# Autodesk Inventor assembly: MOR-20C-6-10
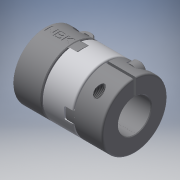
[picture p0: Inventor's stored thumbnail of the model, 180x180]
Saved by Autodesk Inventor 2019 (Build 230136000, 136)
## iProperties
Category: PARTsolutions
Company: NBK
Created: 2024-03-13
Part Number: MOR-20C-6-10
Catalog Web Link: www.cadenas.de
Description: MOR-C-
Vendor: NBK
Document SubType Name: Assembly
Designer: psAdmin
Manufacturer: NBK
Mass: 6.20778 g
Surface Area: 44.699 cm^2
Volume: 6.20778 cm^3
Density: 1 g/cm^3
Title: MOR-20C-6-10
Author: Cadenas PARTsolutions
PSOL_IDENT_0: {$CADENAS_DATA/23d-libs/nbk/motion_control_parts/couplicon_mini/oldham_type/mor/mor_c_asmtab.prj},18
PSOL_IDENT_1: 2 {VTYP=3D},{STYP=ASSTAB},{NB=MOR-20C-6-10},{LINA=MOR-20C-6-10},{NN=MOR-C},{DATE=12.03.2024 08:53:07
PSOL_IDENT_2: },{GEOMDATE=13.12.2021 11:44:02},{VERSION=},{LINEID=240},{WBVAR=D1D2},{WBNUMERIC=}  {NB=MOR-20C-6-10
PSOL_IDENT_3: },{LINA=MOR-20C-6-10},{KT=DUMMY},{CN=MOR-20C},{D1D2=6-10},{A=20},{L=8.8},{W=27.6},{E=12.2},{F=4.4},{
PSOL_IDENT_4: G=7.5},{M=M3},{WT=1.5},{D1D2X1='5-5','5-6','5-6.35','5-8','5-9.525','5-10','6-6','6-6.35','6-8','6-9
PSOL_IDENT_5: .525','6-10','6.35-6.35','6.35-8','6.35-9.525','6.35-10','8-8','8-9.525','8-10','9.525-9.525','9.525
PSOL_IDENT_6: -10','10-10','1/4-1/4','1/4-5/16','1/4-3/8','5/16-5/16','5/16-3/8','3/8-3/8','5-1/4','5-5/16','5-3/8'
PSOL_IDENT_7: ,'6-1/4','6-5/16','6-3/8','6.35-1/4','6.35-5/16','6.35-3/8','8-3/8','9.525-3/8','1/4-8','1/4-9.525','
PSOL_IDENT_8: 1/4-10','5/16-8','5/16-9.525','5/16-10','3/8-10'},{D1=6},{D2=10},{PPATH=mor_c_asmtpl.prj},{CNSORDERN
PSOL_IDENT_9: O=MOR-20C-6-10}
NB: MOR-20C-6-10
NN: MOR-C
NBSYN: $CN.-$D1D2.
LINA: MOR-20C-6-10
CATALOG: NBK (Nabeya Bi-tech Kaisha
CN: MOR-20C
D1D2: 6-10
A: 20
L: 8.8
W: 27.6
E: 12.2
F: 4.4
G: 7.5
M: M3
WT: 1.5
SUPPLIER: NBK
ARTICLENO: MOR-20C-6-10
BOMINFO: MOR-20C-6-10
CREATOR: CADENAS GmbH
## Documents named in this file (4)
- e:\temp\worker_COMMON_2\temp\tmp_7396_62_syEQ4\format_0\MOR-20C-6-10.iam
- e:\temp\worker_COMMON_2\temp\tmp_7396_62_syEQ4\format_0\MOR-20C - 6-10 Hub 1.ipt
- e:\temp\worker_COMMON_2\temp\tmp_7396_62_syEQ4\format_0\MOR-20C  Sleeve.ipt
- e:\temp\worker_COMMON_2\temp\tmp_7396_62_syEQ4\format_0\MOR-20C - 6-10 Hub 2.ipt
## Components (3 placed, 3 different names)
1. MOR-20C - 6-10 Hub 1:1 — p1_p2_XY@1 <-> p2_p1_XY@2, p1_p2_Z@1 <-> p2_p1_Z@2, p1_p2_YZ@1 <-> p2_p1_YZ@2
2. MOR-20C  Sleeve:1 — p1_p2_XY@1 <-> p2_p1_XY@2, p1_p2_Z@1 <-> p2_p1_Z@2, p1_p2_YZ@1 <-> p2_p1_YZ@2, p2_p3_XY@2 <-> p3_p2_XY@3, p2_p3_Z@2 <-> p3_p2_Z@3, p2_p3_YZ@2 <-> p3_p2_YZ@3
3. MOR-20C - 6-10 Hub 2:1 — p2_p3_XY@2 <-> p3_p2_XY@3, p2_p3_Z@2 <-> p3_p2_Z@3, p2_p3_YZ@2 <-> p3_p2_YZ@3
## Relationships (6: Mate 4, Angle 2)
- p1_p2_XY@1 <-> p2_p1_XY@2 [Mate]: MOR-20C - 6-10 Hub 1:1 ↔ MOR-20C  Sleeve:1
- p1_p2_Z@1 <-> p2_p1_Z@2 [Mate]: MOR-20C - 6-10 Hub 1:1 ↔ MOR-20C  Sleeve:1
- p1_p2_YZ@1 <-> p2_p1_YZ@2 [Angle] (0 deg): MOR-20C - 6-10 Hub 1:1 ↔ MOR-20C  Sleeve:1
- p2_p3_XY@2 <-> p3_p2_XY@3 [Mate]: MOR-20C  Sleeve:1 ↔ MOR-20C - 6-10 Hub 2:1
- p2_p3_Z@2 <-> p3_p2_Z@3 [Mate]: MOR-20C  Sleeve:1 ↔ MOR-20C - 6-10 Hub 2:1
- p2_p3_YZ@2 <-> p3_p2_YZ@3 [Angle] (90 deg): MOR-20C  Sleeve:1 ↔ MOR-20C - 6-10 Hub 2:1
